# Autodesk Inventor assembly: viperx_hand_ver2
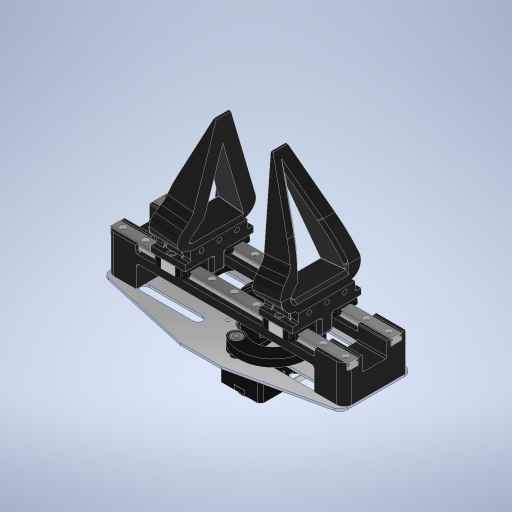
[picture p0: Inventor's stored thumbnail of the model, 512x512]
Saved by Autodesk Inventor 2024.3 (Build 283343010, 343A)
## iProperties
Created: 2025-12-01
Part Number: viperx_hand_ver2
Document SubType Name: Assembly
Designer: kshau
Author: kshau
## Documents named in this file (13)
- C:\Users\kshau\Documents\inventor\Create_ViperX\Create_ViperX_ALOHA\ViperX_hand\viperx_hand_ver2.iam
- C:\Users\kshau\Documents\inventor\Create_ViperX\Create_ViperX_ALOHA\ViperX_hand\bridge_rails_support_ver2.ipt
- C:\Users\kshau\Documents\inventor\Create_ViperX\Create_ViperX_ALOHA\NessesaryParts\SSE2BSZ8-160_STEP_AP203_20250628\SSE2BSZ8-160\SSE2BSZ8-160\SSE2BSZ8-160.iam
- C:\Users\kshau\Documents\inventor\Create_ViperX\Create_ViperX_ALOHA\ViperX_hand\finger_adaptor_ver2.ipt
- C:\Users\kshau\Documents\inventor\Create_ViperX\Create_ViperX_ALOHA\ViperX_hand\rotor_arm_ver2.ipt
- C:\Users\kshau\Documents\inventor\Create_ViperX\Create_ViperX_ALOHA\NessesaryParts\NTN_WA673SA\WA673SA\WA673SA\WA673SA.ipt
- C:\Users\kshau\Documents\inventor\Create_ViperX\Create_ViperX_ALOHA\ViperX_hand\rotor_ver2.ipt
- C:\Users\kshau\Documents\inventor\Create_ViperX\Create_ViperX_ALOHA\NessesaryParts\Bearing36.ipt
- C:\Users\kshau\Documents\inventor\Create_ViperX\Create_ViperX_ALOHA\ViperX_hand\rotor_shim.ipt
- C:\Users\kshau\Documents\inventor\Create_ViperX\Create_ViperX_ALOHA\ViperX_hand\joint_adaptor_plate.ipt
- C:\Users\kshau\Documents\inventor\Create_ViperX\Create_ViperX_ALOHA\Actuator\XM,H-430_idler\XM,H-430_idler\XM,H-430_idler.iam
- C:\Users\kshau\Documents\inventor\Create_ViperX\Create_ViperX_ALOHA\ViperX_hand\finger.ipt
- C:\Users\kshau\Documents\inventor\Create_ViperX\Create_ViperX_ALOHA\ViperX_hand\finger_MIR1.ipt
## Components (23 placed, 12 different names)
1. bridge_rails_support_ver2:1 — 回転:1, 回転:2, 回転:3, 回転:4, 回転:15, 回転:16
2. SSE2BSZ8-160:1 [sub-assembly] — 回転:1, 回転:2, 回転:6, 回転:7
3. SSE2BSZ8-160:2 [sub-assembly] — 回転:3, 回転:4, 回転:5, 回転:8
4. finger_adaptor_ver2:1 — 回転:5, 回転:6, 回転:9, メイト:11, メイト:12, メイト:22, メイト:23, フラッシュ:1
5. finger_adaptor_ver2:2 — 回転:7, 回転:8, メイト:1, メイト:2, 回転:10, フラッシュ:2, メイト:24, メイト:25
6. rotor_arm_ver2:1 — メイト:3, メイト:4, メイト:5, メイト:6, メイト:13, メイト:14, メイト:17, メイト:18
7. WA673SA:1 — メイト:3, メイト:4, 回転:9
8. WA673SA:2 — メイト:5, メイト:6
9. WA673SA:3 — メイト:1, メイト:2
10. rotor_arm_ver2:2 — メイト:7, メイト:8, メイト:9, メイト:10, メイト:15, メイト:16, メイト:19, メイト:20
11. WA673SA:4 — メイト:9, メイト:10, 回転:10
12. WA673SA:5 — メイト:7, メイト:8
13. WA673SA:6 — メイト:11, メイト:12
14. rotor_ver2:1 — 回転:11, 回転:12, 回転:13, 回転:14
15. Bearing36:1 — メイト:19, メイト:20
16. Bearing36:2 — メイト:17, メイト:18
17. Bearing36:3 — メイト:13, メイト:14, 回転:11
18. Bearing36:4 — メイト:15, メイト:16, 回転:12
19. rotor_shim:1 — 回転:13, 回転:14, メイト:21
20. joint_adaptor_plate:1 — 回転:15, 回転:16, メイト:21, 回転:17, 回転:18
21. XM,H-430_idler:1 [sub-assembly] — 回転:17, 回転:18
22. finger:1 — メイト:22, メイト:23, フラッシュ:1
23. finger_MIR1:1 — フラッシュ:2, メイト:24, メイト:25
## Relationships (45: Mate 25, RevoluteJoint 18, Flush 2)
- 回転:1 [RevoluteJoint]: bridge_rails_support_ver2:1 ↔ SSE2BSZ8-160:1
- 回転:2 [RevoluteJoint]: bridge_rails_support_ver2:1 ↔ SSE2BSZ8-160:1
- 回転:3 [RevoluteJoint]: bridge_rails_support_ver2:1 ↔ SSE2BSZ8-160:2
- 回転:4 [RevoluteJoint]: bridge_rails_support_ver2:1 ↔ SSE2BSZ8-160:2
- 回転:5 [RevoluteJoint]: SSE2BSZ8-160:2 ↔ finger_adaptor_ver2:1
- 回転:6 [RevoluteJoint]: SSE2BSZ8-160:1 ↔ finger_adaptor_ver2:1
- 回転:7 [RevoluteJoint]: SSE2BSZ8-160:1 ↔ finger_adaptor_ver2:2
- 回転:8 [RevoluteJoint]: SSE2BSZ8-160:2 ↔ finger_adaptor_ver2:2
- メイト:1 [Mate]: finger_adaptor_ver2:2 ↔ WA673SA:3
- メイト:2 [Mate]: finger_adaptor_ver2:2 ↔ WA673SA:3
- メイト:3 [Mate]: rotor_arm_ver2:1 ↔ WA673SA:1
- メイト:4 [Mate]: rotor_arm_ver2:1 ↔ WA673SA:1
- メイト:5 [Mate]: rotor_arm_ver2:1 ↔ WA673SA:2
- メイト:6 [Mate]: rotor_arm_ver2:1 ↔ WA673SA:2
- 回転:9 [RevoluteJoint]: finger_adaptor_ver2:1 ↔ WA673SA:1
- メイト:7 [Mate]: rotor_arm_ver2:2 ↔ WA673SA:5
- メイト:8 [Mate]: rotor_arm_ver2:2 ↔ WA673SA:5
- メイト:9 [Mate]: rotor_arm_ver2:2 ↔ WA673SA:4
- メイト:10 [Mate]: rotor_arm_ver2:2 ↔ WA673SA:4
- 回転:10 [RevoluteJoint]: finger_adaptor_ver2:2 ↔ WA673SA:4
- メイト:11 [Mate]: finger_adaptor_ver2:1 ↔ WA673SA:6
- メイト:12 [Mate]: finger_adaptor_ver2:1 ↔ WA673SA:6
- メイト:13 [Mate]: rotor_arm_ver2:1 ↔ Bearing36:3
- メイト:14 [Mate]: rotor_arm_ver2:1 ↔ Bearing36:3
- メイト:15 [Mate]: rotor_arm_ver2:2 ↔ Bearing36:4
- メイト:16 [Mate]: rotor_arm_ver2:2 ↔ Bearing36:4
- メイト:17 [Mate]: rotor_arm_ver2:1 ↔ Bearing36:2
- メイト:18 [Mate]: rotor_arm_ver2:1 ↔ Bearing36:2
- メイト:19 [Mate]: rotor_arm_ver2:2 ↔ Bearing36:1
- メイト:20 [Mate]: rotor_arm_ver2:2 ↔ Bearing36:1
- 回転:11 [RevoluteJoint]: rotor_ver2:1 ↔ Bearing36:3
- 回転:12 [RevoluteJoint]: rotor_ver2:1 ↔ Bearing36:4
- 回転:13 [RevoluteJoint]: rotor_ver2:1 ↔ rotor_shim:1
- 回転:14 [RevoluteJoint]: rotor_ver2:1 ↔ rotor_shim:1
- 回転:15 [RevoluteJoint]: bridge_rails_support_ver2:1 ↔ joint_adaptor_plate:1
- 回転:16 [RevoluteJoint]: bridge_rails_support_ver2:1 ↔ joint_adaptor_plate:1
- メイト:21 [Mate]: rotor_shim:1 ↔ joint_adaptor_plate:1
- 回転:17 [RevoluteJoint]: joint_adaptor_plate:1 ↔ XM,H-430_idler:1
- 回転:18 [RevoluteJoint]: joint_adaptor_plate:1 ↔ XM,H-430_idler:1
- メイト:22 [Mate]: finger_adaptor_ver2:1 ↔ finger:1
- メイト:23 [Mate]: finger_adaptor_ver2:1 ↔ finger:1
- フラッシュ:1 [Flush]: finger_adaptor_ver2:1 ↔ finger:1
- フラッシュ:2 [Flush]: finger_adaptor_ver2:2 ↔ finger_MIR1:1
- メイト:24 [Mate]: finger_adaptor_ver2:2 ↔ finger_MIR1:1
- メイト:25 [Mate]: finger_adaptor_ver2:2 ↔ finger_MIR1:1
